# Autodesk Inventor assembly: Z axis motor mount sub-assembly
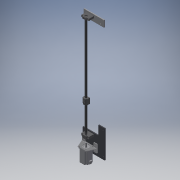
[picture p0: Inventor's stored thumbnail of the model, 180x180]
Saved by Autodesk Inventor 2018 (Build 220112000, 112)
## iProperties
Created: 2018-03-20
Part Number: Z axis motor mount sub-assembly
Document SubType Name: Assembly
Designer: M224826
Author: M224826
## Documents named in this file (6)
- C:\Users\P301319\Documents\GitHub\CNC-Lathe-CAD\CNC Lathe Project\Project Files\Updated Z axis\Z axis motor mount sub-assembly.iam
- C:\Users\P301319\Documents\GitHub\CNC-Lathe-CAD\CNC Lathe Project\Project Files\Updated Z axis\Motor Support Fin.ipt
- C:\Users\P301319\Documents\GitHub\CNC-Lathe-CAD\CNC Lathe Project\Project Files\Updated Z axis\SUPPORT MAIN FRAME MOTOR-BALL SCREW-REV-B.ipt
- C:\Users\P301319\Documents\GitHub\CNC-Lathe-CAD\CNC Lathe Project\Project Files\Servo Motor\Servo Motor.iam
- C:\Users\P301319\Documents\GitHub\CNC-Lathe-CAD\CNC Lathe Project\Project Files\Updated Z axis\AIS2016\Z-AxisLong-Shaft-Final.iam
- C:\Users\P301319\Documents\GitHub\CNC-Lathe-CAD\CNC Lathe Project\Project Files\Updated Z axis\Ball screw right hand support.ipt
## Components (5 placed, 5 different names)
1. Motor Support Fin:1 — Mate:3, Mate:5, Angle:1, Mate:6, Mate:7, Mate:8
2. SUPPORT MAIN FRAME MOTOR-BALL SCREW-REV-B:1 — Flush:1, Flush:2, Flush:3, Mate:3, Mate:6, Mate:7, Mate:9, Mate:10, Mate:11
3. Servo Motor:1 [sub-assembly] — Mate:5, Angle:1, Mate:8
4. Z-AxisLong-Shaft-Final:1 [sub-assembly] — Mate:9, Mate:10, Mate:11, Mate:14, Mate:15, Mate:16
5. Ball screw right hand support:1 — Mate:14, Mate:15, Mate:16
## Relationships (15: Mate 11, Flush 3, Angle 1)
- Flush:1: SUPPORT MAIN FRAME MOTOR-BALL SCREW-REV-B:1
- Flush:2: SUPPORT MAIN FRAME MOTOR-BALL SCREW-REV-B:1
- Flush:3: SUPPORT MAIN FRAME MOTOR-BALL SCREW-REV-B:1
- Mate:3: Motor Support Fin:1 ↔ SUPPORT MAIN FRAME MOTOR-BALL SCREW-REV-B:1
- Mate:5: Motor Support Fin:1 ↔ Servo Motor:1
- Angle:1 (90 deg): Motor Support Fin:1 ↔ Servo Motor:1
- Mate:6: Motor Support Fin:1 ↔ SUPPORT MAIN FRAME MOTOR-BALL SCREW-REV-B:1
- Mate:7: Motor Support Fin:1 ↔ SUPPORT MAIN FRAME MOTOR-BALL SCREW-REV-B:1
- Mate:8: Motor Support Fin:1 ↔ Servo Motor:1
- Mate:9: SUPPORT MAIN FRAME MOTOR-BALL SCREW-REV-B:1 ↔ Z-AxisLong-Shaft-Final:1
- Mate:10: SUPPORT MAIN FRAME MOTOR-BALL SCREW-REV-B:1 ↔ Z-AxisLong-Shaft-Final:1
- Mate:11: SUPPORT MAIN FRAME MOTOR-BALL SCREW-REV-B:1 ↔ Z-AxisLong-Shaft-Final:1
- Mate:14: Z-AxisLong-Shaft-Final:1 ↔ Ball screw right hand support:1
- Mate:15: Z-AxisLong-Shaft-Final:1 ↔ Ball screw right hand support:1
- Mate:16: Z-AxisLong-Shaft-Final:1 ↔ Ball screw right hand support:1
